# Autodesk Inventor assembly: STP16XL031-A-P10_MIR
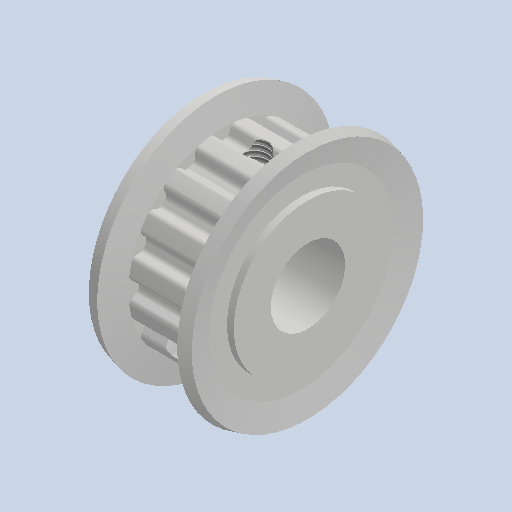
[picture p0: Inventor's stored thumbnail of the model, 512x512]
Saved by Autodesk Inventor 2024.1 (Build 281209000, 209)
## iProperties
Category: PARTsolutions
Company: MISUMI
Created: 2023-12-09
Part Number: STP16XL031-A-P10_MIR
Catalog Web Link: www.cadenas.de
Description: ATP__XL025, ATP__XL031, ATP__ XL037, ATP__XL050, BTP__XL025, BTP__XL031, BTP__XL037, BTP__XL050, KTP__XL025, KTP__XL031, KTP__ XL037, KTP__XL050, NTP__XL025, NTP__XL031, NTP__ XL037, NTP__XL050, MTP__XL025, MTP__ XL037, MTP__XL050, MTPB__XL025, MTPB__ XL037, MTPB__XL050, MTPP__XL025, MTPP__ XL037, MTPP__XL050, STP__XL025, STP__XL031, STP__ XL037, STP__XL050, KATP__XL025, KATP__XL031, KATP__ XL037, KATP__XL050, KKTP__XL025, KKTP__XL031, KKTP__ XL037, KKTP__XL050-Timing Pulleys XL Type
Vendor: MISUMI
Document SubType Name: Assembly
Designer: haruy
Manufacturer: MISUMI
Mass: 6.10935 g
Surface Area: 41.0191 cm^2
Volume: 6.10935 cm^3
Density: 1 g/cm^3
Title: STP16XL031-A-P10
Author: Cadenas PARTsolutions
Comments: Timing Pulleys XL Type
PSOL_IDENT_0: {$CADENAS_DATA/23d-libs/misumi/metric/51_timing_pulleys/mtp_xl_asmtab.prj},894 {VTYP=3D},{STYP=ASSTA
PSOL_IDENT_1: B},{NB=STP16XL031-A-P10},{LINA=STP16XL031-A-P10},{NN=ATP__XL025, ATP__XL031, ATP__ XL037, ATP__XL050
PSOL_IDENT_2: , BTP__XL025, BTP__XL031, BTP__XL037, BTP__XL050, KTP__XL025, KTP__XL031, KTP__ XL037, KTP__XL050, N
PSOL_IDENT_3: TP__XL025, NTP__XL031, NTP__ XL037, NTP__XL050, MTP__XL025, MTP__ XL037, MTP__XL050, MTPB__XL025, MT
PSOL_IDENT_4: PB__ XL037, MTPB__XL050, MTPP__XL025, MTPP__ XL037, MTPP__XL050, STP__XL025, STP__XL031, STP__ XL037
PSOL_IDENT_5: , STP__XL050, KATP__XL025, KATP__XL031, KATP__ XL037, KATP__XL050, KKTP__XL025, KKTP__XL031, KKTP__
PSOL_IDENT_6: XL037, KKTP__XL050},{DATE=06.01.2023 09:05:48},{GEOMDATE=06.01.2023 09:05:40},{VERSION=},{LINEID=30}
PSOL_IDENT_7: ,{WBVAR=MATP,ST,TNW,PS,SBS,DD,Z,J,Q,R,S,T,ALT1,ALT2,M,QSC,QFC,QTC,ALT3,K,KSC,KFC,KTC,ALT4,ZM,ZSC,ZFC
PSOL_IDENT_8: ,ZTC,ALT5,ALT6,ALT7,FC,ALT8,SRG,ALT9,BTC,TL,ALT10,TPC,ALT11,BC,ALT12,SLH,ALT13,BN},{WBNUMERIC=DD,Z,J
PSOL_IDENT_9: ,Q,R,S,T,QSC,QFC,QTC,K,KSC,KFC,KTC,ZSC,ZFC,ZTC,FC,SRG,BTC,TL,BC,SLH,BN}  {NB=STP16XL031-A-P10},{LINA=
PSOL_IDENT_10: STP16XL031-A-P10},{KT=DUMMY},{PN=STP16XL031-A-P10},{TYPE=STP},{MATP=SUS304},{MATPALG= 'A2017','Alumi
PSOL_IDENT_11: num Alloy 2000 series','S45C','1045 Carbon Steel Equivalent','SUS304','SUS304', 'A6000', '6000 Serie
PSOL_IDENT_12: s Aluminum Alloy' },{ST=-},{STALG= '-','-' },{NT=16},{TNW=XL031},{TNWALG= 'XL025','XL031','XL037','X
PSOL_IDENT_13: L050' },{BW=7.9mm (5/16inch)},{PS=A},{PSALG= 'A','B' },{SBS=P},{SBSALG= 'H','Round Hole','P','Round
PSOL_IDENT_14: Hole + Tap','N','New JIS Keywayed Bore + Tap (Standard)','NK','New JIS Keywayed Bore + Tap (width 4.
PSOL_IDENT_15: 0mm, height 1.8mm)','C','Old JIS Keywayed Bore + Tap','V','Stepped Hole','Y','Both Ends Stepped Hole'
PSOL_IDENT_16: ,'WB','Double Stepped Hole' },{DD=10.00},{DDALG=[5:6/1],6.35,[7:12/1],12.7,[13:13/1]},{DDHA=[5:6/1],
PSOL_IDENT_17: 6.35,[7:12/1],12.7,[13:16/1]},{DDPA=[5:6/1],6.35,[7:12/1],12.7,[13:13/1]},{DDNA=[8:8/1],[10:13/1]},{
PSOL_IDENT_18: DDNK=[10:10/1]},{DDCA=[10,12]},{DDVA=[5:6/1],6.35,[7:12/1],12.7,[13:14/1]},{DDY=[5:14/1]},{DDWB=[5:1
PSOL_IDENT_19: 2/1]},{DDHB=},{DDPB=},{DDNB=},{DDCB=},{DDVFB=},{Z=0},{ZALG=[0]},{ZMIN=12.000},{ZAMAX=16.000},{ZBMAX=
PSOL_IDENT_20: 0.000},{DDZ=10.000},{J=0.0},{JALG=[0]},{JMIN=2.000},{JMAX=12.000},{JPN=},{Q=0},{QALG=[0]},{QRMIN=12.
PSOL_IDENT_21: 000},{QRMAX=16},{WBQMIN=14.000},{R=0},{RALG=[0]},{WBRMAX=-2.000},{S=0.0},{SALG=[0]},{SMAX=8},{T=0.0}
PSOL_IDENT_22: ,{TALG=[0]},{TMAX=8},{SBSPN=-P10},{A=9.0},{W=14.0},{L=0},{PD=25.87},{OD=25.36},{D=0},{DALG=17.000},{
PSOL_IDENT_23: DE=20},{F=32},{E=20},{TT=1.6},{BBK=0.000},{TTK=0.0},{ALT1=},{ALT1ALG= '','w/o KC90 (Set Screw Angle)'
PSOL_IDENT_24: ,'KC90','with KC90 (Set Screw Angle)' },{ANG=112.500},{ALT1PN=},{ALT2=},{ALT2ALG= '','Not applicable'
PSOL_IDENT_25: },{M=N/A},{MALG= 'N/A' },{MFTALG= 'N/A' },{MSALG= 'N/A' },{M3D=0.000},{KDML=0.000},{ML=0.000},{MUL=
PSOL_IDENT_26: 0.000},{PITCH=0.000},{QSC=0.0},{QSCALG=0},{QFC=0.0},{QFCALG=0},{QTC=0.0},{QTCALG=0},{QPCDMIN=0.000},
PSOL_IDENT_27: {QPCDMINALG=0.000},{QPCDMAX=16.000},{ALT2PN=},{TAP=0.000},{ALT3=},{ALT3ALG= '','Not applicable' },{K=
PSOL_IDENT_28: 0.0},{KALG=0},{KMIN=4.000},{KFTMAX=0.000},{KSMAX=0.000},{KSC=0.0},{KSCALG=0},{KFC=0.0},{KFCALG=0},{K
PSOL_IDENT_29: TC=0.0},{KTCALG=0},{KSCMIN=14.000},{KPCDMIN=14.000},{KPCDMAX=16.000},{ALT3PN=},{ALT4=},{ALT4ALG= '','
PSOL_IDENT_30: Not applicable' },{ALT4MIN=20.500},{ALT4MAX=9.500},{ZM=N/A},{ZMALG= 'N/A' },{ZMFTALG= 'N/A' },{ZMSAL
PSOL_IDENT_31: G= 'N/A' },{ZMDD1=0.0},{ZMDD2=0.0},{ZMHH=0.0},{ZSC=0.0},{ZSCALG=[0]},{ZFC=0.0},{ZFCALG=[0]},{ZTC=0.0
PSOL_IDENT_32: },{ZTCALG=[0]},{ZPCDMIN=0.000},{ZPCDMINALG=0.000},{ZPCDMAX=16.000},{ALT4PN=},{ALT5=},{ALT5ALG= '','w
PSOL_IDENT_33: /o Flange not Attached','NFC','with NFC (Flange not Attached)' },{ALT5PN=},{ALT6=},{ALT6ALG= '','w/o
PSOL_IDENT_34: Flange Attached on One Side Only','RFC','with RFC (Flange Attached on The Boss Side Only)','LFC','w
PSOL_IDENT_35: ith LFC (Flange Attached on The Opposite Side Only)' },{ALT6PN=},{ALT7=},{ALT7ALG= '','w/o FC (Flang
PSOL_IDENT_36: e Cut)','FC','with FC (Flange Cut)' },{FC=0.0},{FCALG=0},{FCMIN=26.5},{FCMAX=30.0},{ALT7PN=},{ALT8=}
PSOL_IDENT_37: ,{ALT8ALG= '','Not applicable' },{ALT8ALGALG=16.000},{ALT8DD2=0.000},{ALT8MM=0.000},{ALT8NN=0.000},{
PSOL_IDENT_38: QC=0.000},{KC=0.000},{ZC=0.000},{SRG=0.0},{SRGALG=[0]},{SRGMAX=0.000},{DD2=0.0},{MM=0.00},{NN=0.00},
PSOL_IDENT_39: {ALT8PN=},{ALT9=},{ALT9ALG= '','w/o BTC (Taper for Bearing Holder)','BTC','with BTC (Taper for Beari
PSOL_IDENT_40: ng Holder)' },{BTC9=11.000},{TL9=1.000},{BTC=0},{BTCALG=[0]},{TL=0.0},{TLALG=0},{TLMIN=1.000},{TLMAX=
PSOL_IDENT_41: -14.500},{BTCL=0},{BTCD=0},{ALT9PN=},{WLBCTL=14.000},{ALT10=},{ALT10ALG= '','w/o TPC (Tapped Hole Di
PSOL_IDENT_42: mension)','TPC','with TPC (Tapped Hole Dimension)' },{TPC=N/A},{TPCALG= 'N/A' },{TPCM=4.000},{ALT10P
PSOL_IDENT_43: N=},{ALT11=},{ALT11ALG= '','Not applicable' },{BC=0.0},{BCALG=0},{BCMIN=7},{BCMAX=-14.5},{M1WBC=7},{
PSOL_IDENT_44: ALT11PN=},{KTT=7.68},{ALT12=},{ALT12ALG= '','w/o SLH (Set Screw Length)','SLH','with SLH (Set Screw
PSOL_IDENT_45: Length)' },{SLH=0},{SLHALG=[0]},{ALT12PN=},{ALT13=},{ALT13ALG= '', 'Not applicable' },{BN=0.0},{BNAL
PSOL_IDENT_46: G=0},{BNMIN=-13.5},{BNMAX=-4},{ALT13PN=},{AC=M4x3},{M1=4.000},{M1L=3.000},{KEYA=1.000},{KEYB=0.000},
PSOL_IDENT_47: {KEYM=1.000},{PPATH=mtp_xl/mtp_xl_asmtpl.prj}
NB: STP16XL031-A-P10
NN: 0
NT: 16
NBSYN: $PN.
LINA: STP16XL031-A-P10
CATALOG: Misumi
PN: STP16XL031-A-P10
MATP: SUS304
ST: -
TNW: XL031
BW: 7.9mm (5/16inch)
PS: A
SBS: Round Hole + Tap
DD: 10
Z: 0
J: 0
Q: 0
R: 0
S: 0
T: 0
A: 9
W: 14
L: 0
PD: 25.87
OD: 25.36
D: 0
F: 32
E: 20
TT: 1.6
ALT1: w/o KC90 (Set Screw Angle)
ALT2: Not applicable
M: N/A
QSC: 0
QFC: 0
QTC: 0
ALT3: Not applicable
K: 0
KSC: 0
KFC: 0
KTC: 0
ALT4: Not applicable
ZM: N/A
ZMDD1: 0
ZMDD2: 0
ZMHH: 0
ZSC: 0
ZFC: 0
ZTC: 0
ALT5: w/o Flange not Attached
ALT6: w/o Flange Attached on One Side Only
ALT7: w/o FC (Flange Cut)
FC: 0
ALT8: Not applicable
SRG: 0
DD2: 0
MM: 0
ALT9: w/o BTC (Taper for Bearing Holder)
BTC: 0
TL: 0
BTCL: 0
BTCD: 0
ALT10: w/o TPC (Tapped Hole Dimension)
TPC: N/A
ALT11: Not applicable
BC: 0
ALT12: w/o SLH (Set Screw Length)
SLH: 0
ALT13: Not applicable
BN: 0
AC: M4x3
SUPPLIER: MISUMI
ARTICLENO: STP16XL031-A-P10
BOMINFO: STP16XL031-A-P10
CREATOR: CADENAS GmbH
## Documents named in this file (3)
- C:\Users\haruy\OneDrive - Kyushu University\KURT_工房共有\2023~2024\ハード\CAD\2024NHK\000_parts\タイミングベルト\STP16XL031-A-P10_Autodesk_Inventor_2024_20231209 (1)\AIS2024\STP16XL031-A-P10_MIR.iam
- C:\Users\haruy\OneDrive - Kyushu University\KURT_工房共有\2023~2024\ハード\CAD\2024NHK\000_parts\タイミングベルト\STP16XL031-A-P10_Autodesk_Inventor_2024_20231209 (1)\AIS2024\STP16XL031-A-P10_b_MIR.ipt
- C:\Users\haruy\OneDrive - Kyushu University\KURT_工房共有\2023~2024\ハード\CAD\2024NHK\000_parts\タイミングベルト\STP16XL031-A-P10_Autodesk_Inventor_2024_20231209 (1)\AIS2024\SET-SCREW4-3_MIR.ipt
## Components (3 placed, 2 different names)
1. STP16XL031-A-P10_b_MIR:1 — to_screw1_Z@1 <-> CP_Z@2, to_screw2_Z@1 <-> CP_Z@3
2. SET-SCREW4-3_MIR:1 — to_screw1_Z@1 <-> CP_Z@2
3. SET-SCREW4-3_MIR:2 — to_screw2_Z@1 <-> CP_Z@3
## Relationships (2: Mate 2)
- to_screw1_Z@1 <-> CP_Z@2 [Mate]: STP16XL031-A-P10_b_MIR:1 ↔ SET-SCREW4-3_MIR:1
- to_screw2_Z@1 <-> CP_Z@3 [Mate]: STP16XL031-A-P10_b_MIR:1 ↔ SET-SCREW4-3_MIR:2
